# Autodesk Inventor assembly: Motor Med Gear
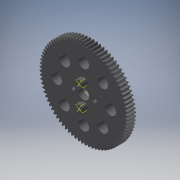
[picture p0: Inventor's stored thumbnail of the model, 180x180]
Saved by Autodesk Inventor 2016 (Build 200138000, 138)
## iProperties
Created: 2015-12-14
Part Number: Motor Med Gear
Document SubType Name: Assembly
Designer: tbloo
Author: tbloo
## Documents named in this file (4)
- C:\Users\tbloo\Documents\GitHub\phi_robotics\3d-models\FTC_Tetrix_KOP_Block_Party\Tim Bloot Designs\JAr JaR Bot\Motor Med Gear.iam
- C:\Users\tbloo\Documents\GitHub\phi_robotics\3d-models\FTC_Tetrix_KOP_Block_Party\Tetrix_Kit_FTC\Autodesk Inventor Files\tetrix_gear-med.ipt
- C:\Users\tbloo\Documents\GitHub\phi_robotics\3d-models\FTC_Tetrix_KOP_Block_Party\Tetrix_Kit_FTC\Autodesk Inventor Files\tetrix_maxle_lock.iam
- C:\Users\tbloo\Documents\GitHub\phi_robotics\3d-models\FTC_Tetrix_KOP_Block_Party\Tetrix_Kit_FTC\Autodesk Inventor Files\tetrix_screw.ipt
## Components (4 placed, 3 different names)
1. tetrix_gear-med:1 — Rigid:2, Rigid:3, Rigid:4
2. tetrix_maxle_lock:1 [sub-assembly] — Rigid:2
3. tetrix_screw:1 — Rigid:3
4. tetrix_screw:2 — Rigid:4
## Relationships (3: WeldJoint 3)
- Rigid:2 [WeldJoint]: tetrix_gear-med:1 ↔ tetrix_maxle_lock:1
- Rigid:3 [WeldJoint]: tetrix_gear-med:1 ↔ tetrix_screw:1
- Rigid:4 [WeldJoint]: tetrix_gear-med:1 ↔ tetrix_screw:2
